# Autodesk Inventor assembly: PS20020
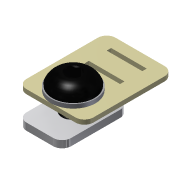
[picture p0: Inventor's stored thumbnail of the model, 180x180]
Saved by Autodesk Inventor 2014 (Build 180170000, 170)
## iProperties
Created: 2013-05-31
Part Number: PS20020
Document SubType Name: Assembly
Designer: Edward
Mass: 2.88191 g
Surface Area: 15.4013 cm^2
Volume: 0.765461 cm^3
Density: 3.76494 g/cm^3
Description: Belt Clip Assembly
Author: Edward
Title: Belt Clip Assembly
Subject: Shapeoko 2
## Documents named in this file (5)
- C:\Users\Edward\Documents\GitHub\Shapeoko_2\Autodesk_Inventor_Project\PS20020.iam
- C:\Users\Edward\Documents\GitHub\Shapeoko_2\Autodesk_Inventor_Project\26051-01.ipt
- C:\Users\Edward\Documents\GitHub\Shapeoko_2\Autodesk_Inventor_Project\PS20003.ipt
- C:\Users\Edward\Documents\GitHub\Shapeoko_2\Autodesk_Inventor_Project\25287-02.ipt
- C:\Users\Edward\Documents\GitHub\Shapeoko_2\Autodesk_Inventor_Project\26016-01.ipt
## Components (4 placed, 4 different names)
1. 26051-01:1 — Insert:2, Insert:3, Angle:1
2. PS20003:1 — Insert:1
3. 25287-02:1 — Insert:1, Insert:2
4. 26016-01:1 — Insert:3, Angle:1
## Relationships (4: Insert 3, Angle 1)
- Insert:1: PS20003:1 ↔ 25287-02:1
- Insert:2: 26051-01:1 ↔ 25287-02:1
- Insert:3 (3 mm): 26051-01:1 ↔ 26016-01:1
- Angle:1 (0 deg): 26051-01:1 ↔ 26016-01:1
